# Autodesk Inventor assembly: final_assembly_camera_holder_filleted
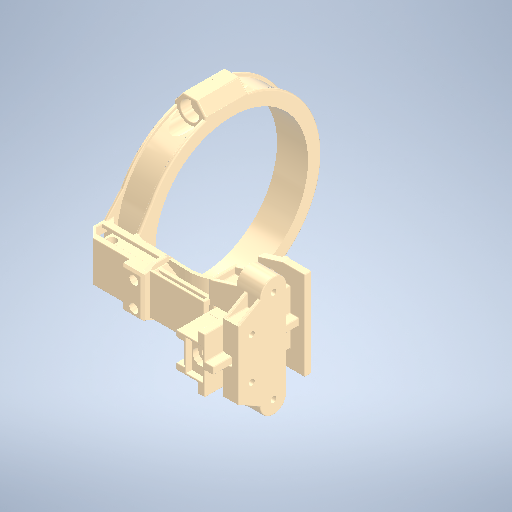
[picture p0: Inventor's stored thumbnail of the model, 512x512]
Saved by Autodesk Inventor 2025 (Build 290162010, 162A)
## iProperties
Created: 2023-09-11
Part Number: final_assembly_camera_holder_filleted
Document SubType Name: Assembly
Designer: caubeeluck
Author: caubeeluck
## Documents named in this file (6)
- D:\Projects\Archived\Misc\github\autoclean\AutoClean\cad_files\camera_holder\final_assembly_camera_holder_filleted.iam
- D:\Projects\Archived\Misc\github\autoclean\AutoClean\cad_files\camera_holder\final_assembly_camera_holder_filleted1.ipt
- D:\Projects\Archived\Misc\github\autoclean\AutoClean\cad_files\camera_holder\final_assembly_camera_holder_filleted2.ipt
- D:\Projects\Archived\Misc\github\autoclean\AutoClean\cad_files\camera_holder\final_assembly_camera_holder_filleted3.ipt
- D:\Projects\Archived\Misc\github\autoclean\AutoClean\cad_files\camera_holder\final_assembly_camera_holder_filleted4.ipt
- D:\Projects\Archived\Misc\github\autoclean\AutoClean\cad_files\camera_holder\final_assembly_camera_holder_filleted5.ipt
## Components (5 placed, 5 different names)
1. final_assembly_camera_holder_filleted1:1 — Mate:1, Mate:2, Mate:3, Mate:4, Mate:5
2. final_assembly_camera_holder_filleted2:1 — Mate:4, Mate:5, Mate:7, Mate:8, Mate:9, Mate:10
3. final_assembly_camera_holder_filleted3:1 — Mate:6, Mate:7, Mate:10
4. final_assembly_camera_holder_filleted4:1 — Mate:1, Mate:2, Mate:3
5. final_assembly_camera_holder_filleted5:1 — Mate:6, Mate:8, Mate:9
## Relationships (10: Mate 10)
- Mate:1: final_assembly_camera_holder_filleted1:1 ↔ final_assembly_camera_holder_filleted4:1
- Mate:2: final_assembly_camera_holder_filleted1:1 ↔ final_assembly_camera_holder_filleted4:1
- Mate:3: final_assembly_camera_holder_filleted1:1 ↔ final_assembly_camera_holder_filleted4:1
- Mate:4: final_assembly_camera_holder_filleted1:1 ↔ final_assembly_camera_holder_filleted2:1
- Mate:5: final_assembly_camera_holder_filleted1:1 ↔ final_assembly_camera_holder_filleted2:1
- Mate:6: final_assembly_camera_holder_filleted3:1 ↔ final_assembly_camera_holder_filleted5:1
- Mate:7: final_assembly_camera_holder_filleted2:1 ↔ final_assembly_camera_holder_filleted3:1
- Mate:8: final_assembly_camera_holder_filleted2:1 ↔ final_assembly_camera_holder_filleted5:1
- Mate:9: final_assembly_camera_holder_filleted2:1 ↔ final_assembly_camera_holder_filleted5:1
- Mate:10: final_assembly_camera_holder_filleted2:1 ↔ final_assembly_camera_holder_filleted3:1
